# Autodesk Inventor assembly: WalkDetection-V1
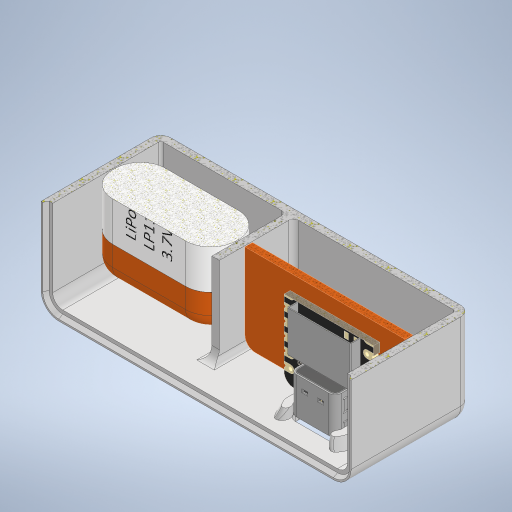
[picture p0: Inventor's stored thumbnail of the model, 512x512]
Saved by Autodesk Inventor 2024.3 (Build 283343000, 343)
## iProperties
Created: 2024-11-30
Part Number: WalkDetection-V1
Document SubType Name: Assembly
Designer: ASUS TUF
Author: ASUS TUF
## Documents named in this file (4)
- C:\Users\ASUS TUF\Documents\Inventor\ParkinsonDetection\WalkDetection-V1.iam
- C:\Users\ASUS TUF\Documents\Inventor\ParkinsonDetection\Case-V1.ipt
- C:\Users\ASUS TUF\Documents\Inventor\ParkinsonDetection\PCB.iam
- C:\Users\ASUS TUF\Documents\Inventor\ParkinsonDetection\LP112527-3.7V650mAh\LP112527-3.7V650mAh\LP112527-3.7V650mAh.ipt
## Components (3 placed, 3 different names)
1. Case-V1:1 — Mate:5, Flush:1, Tangent:4, Tangent:3, Mate:3, Angle:1, Mate:6
2. PCB:1 [sub-assembly] — Mate:5, Flush:1, Mate:3, Mate:4
3. LP112527-3.7V650mAh:1 — Tangent:4, Tangent:3, Mate:4, Angle:1, Mate:6
## Relationships (8: Mate 4, Tangent 2, Flush 1, Angle 1)
- Mate:5 (0.2 mm): Case-V1:1 ↔ PCB:1
- Flush:1: Case-V1:1 ↔ PCB:1
- Tangent:4 (0.2 mm): Case-V1:1 ↔ LP112527-3.7V650mAh:1
- Tangent:3 (0.2 mm): Case-V1:1 ↔ LP112527-3.7V650mAh:1
- Mate:3 (0.2 mm): Case-V1:1 ↔ PCB:1
- Mate:4 (1.9 mm): PCB:1 ↔ LP112527-3.7V650mAh:1
- Angle:1 (0 deg): Case-V1:1 ↔ LP112527-3.7V650mAh:1
- Mate:6: Case-V1:1 ↔ LP112527-3.7V650mAh:1
